# Autodesk Inventor assembly: xy-mount-asm
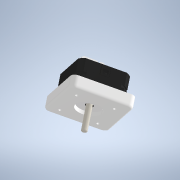
[picture p0: Inventor's stored thumbnail of the model, 180x180]
Saved by Autodesk Inventor 2020 (Build 240168000, 168)
## iProperties
Created: 2021-03-01
Part Number: xy-mount-asm
Document SubType Name: Assembly
Designer: AOB
Mass: 267.413 g
Surface Area: 393.147 cm^2
Volume: 52.4257 cm^3
Density: 5.1008 g/cm^3
Author: AOB
## Documents named in this file (7)
- C:\Users\marti\Documents\Inventor\ProjectBoron\Boron Ultima\xy-mount-asm.iam
- C:\Users\marti\Documents\Inventor\ProjectBoron\Boron Ultima\xy-mount-bottom.ipt
- C:\Users\marti\Documents\Inventor\ProjectBoron\Boron Ultima\xy-mount-tp.ipt
- C:\Users\marti\Documents\Inventor\ProjectBoron\Boron Ultima\lm8uu-graphite.ipt
- C:\Users\marti\Documents\Inventor\ProjectBoron\Boron Ultima\gantry motor mount.ipt
- C:\Users\marti\Documents\Inventor\ProjectBoron\Boron Vega\695zz bearing.ipt
- C:\Users\marti\Documents\Inventor\ProjectBoron\Boron Ultima\NEMA17 pancake motor (23mm).iam
## Components (7 placed, 6 different names)
1. xy-mount-bottom:1 — Flush:1, Cylindrical:1, Cylindrical:2, Mate:1, Flush:3, Mate:2, Mate:3, Flush:4, Mate:10, Mate:9
2. 695zz bearing:1 — Flush:2, Cylindrical:2
3. 695zz bearing:2 — Flush:1, Cylindrical:1
4. xy-mount-tp:1 — Mate:1, Flush:3, Mate:4, Flush:2
5. lm8uu-graphite:1 — Mate:2, Mate:3, Mate:4, Mate:8
6. gantry motor mount:1 — Flush:4, Mate:10, Mate:9, Mate:6, Mate:7, Mate:8
7. NEMA17 pancake motor (23mm):1 [sub-assembly] — Mate:6, Mate:7
## Relationships (16: Mate 9, Flush 4, CylindricalJoint 2, Angle 1)
- Flush:1: xy-mount-bottom:1 ↔ 695zz bearing:2
- Cylindrical:1: xy-mount-bottom:1 ↔ 695zz bearing:2
- Flush:2: 695zz bearing:1 ↔ xy-mount-tp:1
- Cylindrical:2: xy-mount-bottom:1 ↔ 695zz bearing:1
- Mate:1: xy-mount-bottom:1 ↔ xy-mount-tp:1
- Flush:3: xy-mount-bottom:1 ↔ xy-mount-tp:1
- Mate:2: xy-mount-bottom:1 ↔ lm8uu-graphite:1
- Mate:3: xy-mount-bottom:1 ↔ lm8uu-graphite:1
- Mate:4: xy-mount-tp:1 ↔ lm8uu-graphite:1
- Flush:4: xy-mount-bottom:1 ↔ gantry motor mount:1
- Mate:10 (-10 mm): xy-mount-bottom:1 ↔ gantry motor mount:1
- Mate:9 (23.5 mm): xy-mount-bottom:1 ↔ gantry motor mount:1
- Mate:6: gantry motor mount:1 ↔ NEMA17 pancake motor (23mm):1
- Mate:7: gantry motor mount:1 ↔ NEMA17 pancake motor (23mm):1
- [Angle] (90 deg): lm8uu-graphite:1 ↔ NEMA17 pancake motor (23mm):1
- Mate:8: lm8uu-graphite:1 ↔ gantry motor mount:1
